# Autodesk Inventor assembly: Motorwheel
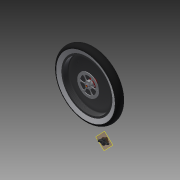
[picture p0: Inventor's stored thumbnail of the model, 180x180]
Saved by Autodesk Inventor 2016 (Build 200138000, 138)
## iProperties
Created: 2015-06-04
Part Number: Motorwheel
Document SubType Name: Assembly
Designer: Yann
Author: Yann
## Documents named in this file (5)
- C:\Users\Yann\Documents\GitHub\BIKAIR_CAD\Source\Motorwheel\Motorwheel.iam
- C:\Users\Yann\Documents\GitHub\BIKAIR_CAD\Source\Motorwheel\Wheel\wheel.iam
- C:\Users\Yann\Documents\Inventor\Content Center Files\R2016\en-US\DIN 628 SKF(1)\DIN 628 SKF - SKF 3302 A-2RS1.ipt
- C:\Users\Yann\Documents\GitHub\BIKAIR_CAD\Source\Motorwheel\Disk Brake Caliper.ipt
- C:\Users\Yann\Documents\GitHub\BIKAIR_CAD\Source\Motorwheel\Hub_Carrier.ipt
## Components (4 placed, 4 different names)
1. wheel:1 [sub-assembly] — Mate:1, Flush:1, Rotational:1, Flush:2
2. DIN 628 SKF- with seals - 32..A-2RS1, 33..A-2RS1 SKF 3302 A-2RS1:1 — Rotational:1
3. Disk Brake Caliper:1 — Flush:2
4. Hub_Carrier:1 — Flush:3, Flush:4, Flush:5
## Relationships (7: Flush 5, Mate 1, RevoluteJoint 1)
- Mate:1: wheel:1
- Flush:1: wheel:1
- Rotational:1 [RevoluteJoint]: wheel:1 ↔ DIN 628 SKF- with seals - 32..A-2RS1, 33..A-2RS1 SKF 3302 A-2RS1:1
- Flush:2: wheel:1 ↔ Disk Brake Caliper:1
- Flush:3: Hub_Carrier:1
- Flush:4: Hub_Carrier:1
- Flush:5: Hub_Carrier:1
